# Autodesk Inventor assembly: 組合窗
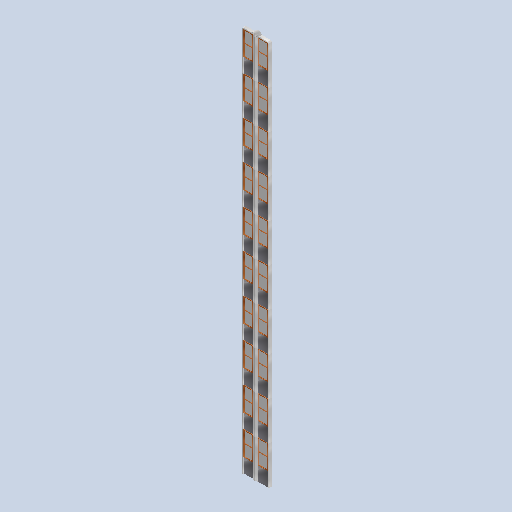
[picture p0: Inventor's stored thumbnail of the model, 512x512]
Saved by Autodesk Inventor 2024.2 (Build 282272000, 272)
## iProperties
Created: 2024-06-01
Part Number: 組合窗
Document SubType Name: Assembly
Designer: User
Author: User
## Documents named in this file (5)
- C:\Users\User\OneDrive - 國立中山大學\桌面\創客基礎\final_project\組合窗.iam
- C:\Users\User\OneDrive - 國立中山大學\桌面\創客基礎\final_project\窗.ipt
- C:\Users\User\OneDrive - 國立中山大學\桌面\創客基礎\final_project\窗間柱.ipt
- C:\Users\User\OneDrive - 國立中山大學\桌面\創客基礎\final_project\窗側柱.ipt
- C:\Users\User\OneDrive - 國立中山大學\桌面\創客基礎\final_project\窗頂.ipt
## Components (51 placed, 4 different names)
1. 窗頂:1 — 貼合:5, 齊平:9, 相切:1
2. 窗:1 — 齊平:1, 貼合:1, 齊平:2, 貼合:3, 齊平:5, 齊平:6
3. 窗間柱:1 — 齊平:1, 貼合:1, 齊平:2, 貼合:2, 齊平:3, 齊平:4, 貼合:5, 齊平:9
4. 窗側柱:2 — 貼合:3, 齊平:5, 齊平:6
5. 窗:2 — 貼合:2, 齊平:3, 齊平:4, 貼合:4, 齊平:7, 齊平:8
6. 窗側柱:1 — 貼合:4, 齊平:7, 齊平:8, 相切:1
7. 窗:3
8. 窗間柱:2
9. 窗側柱:3
10. 窗:4
11. 窗側柱:4
12. 窗:5
13. 窗間柱:3
14. 窗側柱:5
15. 窗:6
16. 窗側柱:6
17. 窗:7
18. 窗間柱:4
19. 窗側柱:7
20. 窗:8
21. 窗側柱:8
22. 窗:9
23. 窗間柱:5
24. 窗側柱:9
25. 窗:10
26. 窗側柱:10
27. 窗:11
28. 窗間柱:6
29. 窗側柱:11
30. 窗:12
31. 窗側柱:12
32. 窗:13
33. 窗間柱:7
34. 窗側柱:13
35. 窗:14
36. 窗側柱:14
37. 窗:15
38. 窗間柱:8
39. 窗側柱:15
40. 窗:16
41. 窗側柱:16
42. 窗:17
43. 窗間柱:9
44. 窗側柱:17
45. 窗:18
46. 窗側柱:18
47. 窗:19
48. 窗間柱:10
49. 窗側柱:19
50. 窗:20
51. 窗側柱:20
## Component patterns: (10 elements, first: 窗:1 + 窗間柱:1 + 窗側柱:2 + 窗:2 + 窗側柱:1)
## Relationships (15: Flush 9, Mate 5, Tangent 1)
- 齊平:1 [Flush]: 窗:1 ↔ 窗間柱:1
- 貼合:1 [Mate]: 窗:1 ↔ 窗間柱:1
- 齊平:2 [Flush]: 窗:1 ↔ 窗間柱:1
- 貼合:2 [Mate]: 窗間柱:1 ↔ 窗:2
- 齊平:3 [Flush]: 窗間柱:1 ↔ 窗:2
- 齊平:4 [Flush]: 窗間柱:1 ↔ 窗:2
- 貼合:3 [Mate]: 窗:1 ↔ 窗側柱:2
- 齊平:5 [Flush]: 窗:1 ↔ 窗側柱:2
- 齊平:6 [Flush]: 窗:1 ↔ 窗側柱:2
- 貼合:4 [Mate]: 窗:2 ↔ 窗側柱:1
- 齊平:7 [Flush]: 窗:2 ↔ 窗側柱:1
- 齊平:8 [Flush]: 窗:2 ↔ 窗側柱:1
- 貼合:5 [Mate]: 窗頂:1 ↔ 窗間柱:1
- 齊平:9 [Flush]: 窗頂:1 ↔ 窗間柱:1
- 相切:1 [Tangent]: 窗頂:1 ↔ 窗側柱:1
